# Autodesk Inventor assembly: rotate bot
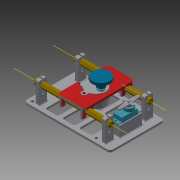
[picture p0: Inventor's stored thumbnail of the model, 180x180]
Saved by Autodesk Inventor 2015 SP2 (Build 190223200, 223)
## iProperties
Created: 2015-05-24
Part Number: rotate bot
Document SubType Name: Assembly
Designer: caleb
Author: caleb
## Documents named in this file (8)
- C:\cygwin64\home\caleb\3d\designs\deep-focus-scanning-adapter\rotate bot.iam
- C:\cygwin64\home\caleb\3d\designs\deep-focus-scanning-adapter\servo micro asm2.iam
- C:\cygwin64\home\caleb\3d\designs\deep-focus-scanning-adapter\stepper motor-cheapo geared.ipt
- C:\cygwin64\home\caleb\3d\designs\deep-focus-scanning-adapter\rotobot rods.ipt
- C:\cygwin64\home\caleb\3d\designs\deep-focus-scanning-adapter\rotobot carriage.ipt
- C:\cygwin64\home\caleb\3d\designs\deep-focus-scanning-adapter\rotobot base.ipt
- C:\cygwin64\home\caleb\3d\designs\deep-focus-scanning-adapter\rotobot pushrod.ipt
- C:\cygwin64\home\caleb\3d\designs\deep-focus-scanning-adapter\turntable.ipt
## Components (7 placed, 7 different names)
1. servo micro asm2:1 [sub-assembly] — Mate:1, Mate:2, Mate:3, Mate:11
2. stepper motor-cheapo geared:1 — Mate:8, Mate:9, Mate:10, Mate:13, Mate:14
3. rotobot rods:1 — Mate:6, Mate:7, Flush:4
4. rotobot carriage:1 — Mate:4, Mate:5, Mate:8, Mate:9, Mate:10, Mate:12
5. rotobot base:1 — Flush:1, Flush:2, Flush:3, Mate:1, Mate:2, Mate:3, Mate:4, Mate:5, Mate:6, Mate:7, Flush:4
6. rotobot pushrod:1 — Mate:11, Mate:12
7. turntable:1 — Mate:13, Mate:14
## Relationships (18: Mate 14, Flush 4)
- Flush:1: rotobot base:1
- Flush:2: rotobot base:1
- Flush:3: rotobot base:1
- Mate:1: servo micro asm2:1 ↔ rotobot base:1
- Mate:2: servo micro asm2:1 ↔ rotobot base:1
- Mate:3: servo micro asm2:1 ↔ rotobot base:1
- Mate:4: rotobot carriage:1 ↔ rotobot base:1
- Mate:5: rotobot carriage:1 ↔ rotobot base:1
- Mate:6: rotobot rods:1 ↔ rotobot base:1
- Mate:7: rotobot rods:1 ↔ rotobot base:1
- Flush:4 (-3 mm): rotobot rods:1 ↔ rotobot base:1
- Mate:8: stepper motor-cheapo geared:1 ↔ rotobot carriage:1
- Mate:9: stepper motor-cheapo geared:1 ↔ rotobot carriage:1
- Mate:10: stepper motor-cheapo geared:1 ↔ rotobot carriage:1
- Mate:11: servo micro asm2:1 ↔ rotobot pushrod:1
- Mate:12: rotobot carriage:1 ↔ rotobot pushrod:1
- Mate:13: stepper motor-cheapo geared:1 ↔ turntable:1
- Mate:14: stepper motor-cheapo geared:1 ↔ turntable:1
